# Autodesk Inventor assembly: 4BevelGears
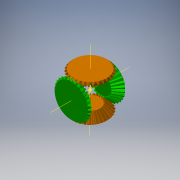
[picture p0: Inventor's stored thumbnail of the model, 180x180]
Saved by Autodesk Inventor 2017 (Build 210142000, 142)
## iProperties
Created: 2018-05-09
Part Number: 4BevelGears
Document SubType Name: Assembly
Designer: skhi8305
Author: skhi8305
## Documents named in this file (2)
- G:\FinalIEDProject\4BevelGears.iam
- G:\FinalIEDProject\BevelGears.iam
## Components (2 placed, 1 different names)
1. BevelGears:1 [sub-assembly] — Rotation:1
2. BevelGears:2 [sub-assembly] — Rotation:1
## Relationships (1: RelateRotation 1)
- Rotation:1 [RelateRotation] (1 ul): BevelGears:1 ↔ BevelGears:2
